# Autodesk Inventor assembly: obudowa
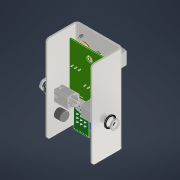
[picture p0: Inventor's stored thumbnail of the model, 180x180]
Saved by Autodesk Inventor 2022 (Build 260153000, 153)
## iProperties
Created: 2021-03-29
Part Number: obudowa
Document SubType Name: Assembly
Designer: Karol
Author: Karol
## Documents named in this file (12)
- E:\gitarowe pedaly\deep blue delay 1\model 3d\obudowa.iam
- E:\gitarowe pedaly\deep blue delay 1\model 3d\dekiel.ipt
- E:\gitarowe pedaly\deep blue delay 1\model 3d\puszka.ipt
- C:\Users\Karol\Documents\Inventor\Content Center Files\R2021\pl-PL\BS EN ISO 7045 H\EN ISO 7045 - M3 x 8 - 4.8 - H(1).ipt
- E:\modele 3d\potencjometry\potencjometr 16 mm pcb V\16mm PCB Pot.ipt
- E:\modele 3d\3pdt\User Library-Footswich_3PDT.ipt
- E:\modele 3d\gniazda jack\amphenol acjm-mvs-2\ACJM-MVS-2.ipt
- E:\modele 3d\gałka na potencjometr\gałka_ze srubka.ipt
- E:\modele 3d\oprawka na led\5mm niklowana\5mm Led bezel nickel (true).ipt
- E:\modele 3d\gniazdo dc\styl boss\DC Power 2.1 Enclosed.ipt
- E:\gitarowe pedaly\3pdt pcb\3pdt kicad\3pdt kicad.ipt
- E:\gitarowe pedaly\deep blue delay 1\model 3d\pcb main.ipt
## Components (19 placed, 11 different names)
1. dekiel:1 — Zestawiające:1, Zestawiające:2, Równoległe:1, Wstawiające:1, Wstawiające:2, Wstawiające:3, Wstawiające:4, Zestawiające:3, Zestawiające:4, Zestawiające:5, Zestawiające:6, Zestawiające:7, Zestawiające:8, Kątowe:1, Zestawiające:9, Zestawiające:10, Zestawiające:11, Zestawiające:12, Zestawiające:13, Zestawiające:14, Kątowe:4, Zestawiające:18, Zestawiające:19, Zestawiające:20, Zestawiające:21, Zestawiające:22
2. puszka:1 — Zestawiające:1, Zestawiające:2, Równoległe:1
3. BS EN ISO 7045 H - Metryczny M3 x 8 - 4.8 - H:1 — Wstawiające:1
4. BS EN ISO 7045 H - Metryczny M3 x 8 - 4.8 - H:2 — Wstawiające:2
5. BS EN ISO 7045 H - Metryczny M3 x 8 - 4.8 - H:3 — Wstawiające:3
6. BS EN ISO 7045 H - Metryczny M3 x 8 - 4.8 - H:4 — Wstawiające:4
7. 16mm PCB Pot:1 — Zestawiające:3, Zestawiające:6, Kątowe:1, Kątowe:2, Zestawiające:15, Zestawiające:26, Zestawiające:27
8. 16mm PCB Pot:2 — Zestawiające:4, Zestawiające:7, Kątowe:2, Kątowe:3, Zestawiające:16
9. 16mm PCB Pot:3 — Zestawiające:5, Zestawiające:8, Kątowe:3, Zestawiające:17, Równoległe:5
10. User Library-Footswich_3PDT:1 — Zestawiające:9, Zestawiające:10, Zestawiające:23, Zestawiające:24, Zestawiające:25
11. ACJM-MVS-2:1 — Zestawiające:12, Zestawiające:14, Równoległe:2, Kątowe:4
12. ACJM-MVS-2:2 — Zestawiające:11, Zestawiające:13, Równoległe:2
13. gałka_ze srubka:1 — Zestawiające:15, Równoległe:4, Zestawiające:18
14. gałka_ze srubka:2 — Zestawiające:16, Równoległe:3, Równoległe:4
15. gałka_ze srubka:3 — Zestawiające:17, Równoległe:3
16. 5mm Led bezel nickel (true):1 — Zestawiające:19, Zestawiające:20
17. DC Power 2.1 Enclosed:1 — Zestawiające:21, Zestawiające:22
18. 3pdt kicad:1 — Zestawiające:23, Zestawiające:24, Zestawiające:25
19. pcb main:1 — Równoległe:5, Zestawiające:26, Zestawiające:27
## Relationships (40: Mate 27, Flush 5, Insert 4, Angle 4)
- Zestawiające:1 [Mate]: dekiel:1 ↔ puszka:1
- Zestawiające:2 [Mate]: dekiel:1 ↔ puszka:1
- Równoległe:1 [Flush] (-4 mm): dekiel:1 ↔ puszka:1
- Wstawiające:1 [Insert]: dekiel:1 ↔ BS EN ISO 7045 H - Metryczny M3 x 8 - 4.8 - H:1
- Wstawiające:2 [Insert]: dekiel:1 ↔ BS EN ISO 7045 H - Metryczny M3 x 8 - 4.8 - H:2
- Wstawiające:3 [Insert]: dekiel:1 ↔ BS EN ISO 7045 H - Metryczny M3 x 8 - 4.8 - H:3
- Wstawiające:4 [Insert]: dekiel:1 ↔ BS EN ISO 7045 H - Metryczny M3 x 8 - 4.8 - H:4
- Zestawiające:3 [Mate]: dekiel:1 ↔ 16mm PCB Pot:1
- Zestawiające:4 [Mate]: dekiel:1 ↔ 16mm PCB Pot:2
- Zestawiające:5 [Mate]: dekiel:1 ↔ 16mm PCB Pot:3
- Zestawiające:6 [Mate]: dekiel:1 ↔ 16mm PCB Pot:1
- Zestawiające:7 [Mate]: dekiel:1 ↔ 16mm PCB Pot:2
- Zestawiające:8 [Mate]: dekiel:1 ↔ 16mm PCB Pot:3
- Kątowe:1 [Angle] (180 deg): dekiel:1 ↔ 16mm PCB Pot:1
- Kątowe:2 [Angle] (180 deg): 16mm PCB Pot:1 ↔ 16mm PCB Pot:2
- Kątowe:3 [Angle] (0 deg): 16mm PCB Pot:2 ↔ 16mm PCB Pot:3
- Zestawiające:9 [Mate]: dekiel:1 ↔ User Library-Footswich_3PDT:1
- Zestawiające:10 [Mate]: dekiel:1 ↔ User Library-Footswich_3PDT:1
- Zestawiające:11 [Mate]: dekiel:1 ↔ ACJM-MVS-2:2
- Zestawiające:12 [Mate]: dekiel:1 ↔ ACJM-MVS-2:1
- Zestawiające:13 [Mate]: dekiel:1 ↔ ACJM-MVS-2:2
- Zestawiające:14 [Mate]: dekiel:1 ↔ ACJM-MVS-2:1
- Równoległe:2 [Flush]: ACJM-MVS-2:1 ↔ ACJM-MVS-2:2
- Kątowe:4 [Angle] (0 deg): dekiel:1 ↔ ACJM-MVS-2:1
- Zestawiające:15 [Mate]: 16mm PCB Pot:1 ↔ gałka_ze srubka:1
- Zestawiające:16 [Mate]: 16mm PCB Pot:2 ↔ gałka_ze srubka:2
- Zestawiające:17 [Mate]: 16mm PCB Pot:3 ↔ gałka_ze srubka:3
- Równoległe:3 [Flush]: gałka_ze srubka:2 ↔ gałka_ze srubka:3
- Równoległe:4 [Flush]: gałka_ze srubka:1 ↔ gałka_ze srubka:2
- Zestawiające:18 [Mate] (1 mm): dekiel:1 ↔ gałka_ze srubka:1
- Zestawiające:19 [Mate]: dekiel:1 ↔ 5mm Led bezel nickel (true):1
- Zestawiające:20 [Mate]: dekiel:1 ↔ 5mm Led bezel nickel (true):1
- Zestawiające:21 [Mate]: dekiel:1 ↔ DC Power 2.1 Enclosed:1
- Zestawiające:22 [Mate]: dekiel:1 ↔ DC Power 2.1 Enclosed:1
- Zestawiające:23 [Mate]: User Library-Footswich_3PDT:1 ↔ 3pdt kicad:1
- Zestawiające:24 [Mate] (0.1 mm): User Library-Footswich_3PDT:1 ↔ 3pdt kicad:1
- Zestawiające:25 [Mate] (0.6 mm): User Library-Footswich_3PDT:1 ↔ 3pdt kicad:1
- Równoległe:5 [Flush]: 16mm PCB Pot:3 ↔ pcb main:1
- Zestawiające:26 [Mate] (-0.6 mm): 16mm PCB Pot:1 ↔ pcb main:1
- Zestawiające:27 [Mate] (-0.25 mm): 16mm PCB Pot:1 ↔ pcb main:1
